# Autodesk Inventor assembly: Ensamble_Base_MX-28
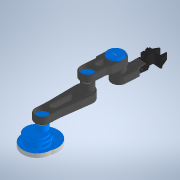
[picture p0: Inventor's stored thumbnail of the model, 180x180]
Saved by Autodesk Inventor 2021 (Build 250183000, 183)
## iProperties
Created: 2022-06-20
Part Number: Ensamble_Base_MX-28
Document SubType Name: Assembly
Designer: Alcatraz
Author: Alcatraz
## Documents named in this file (5)
- F:\Tesis\TESIS\Simulaciones\Movimiento en el plano\Base_MX-28\Ensamble_Base_MX-28.iam
- F:\Tesis\TESIS\Simulaciones\Base_MX28.ipt
- F:\Tesis\TESIS\Simulaciones\Eslabon_1.ipt
- F:\Tesis\TESIS\Simulaciones\Eslabon_2.ipt
- F:\Tesis\TESIS\Simulaciones\Eslabon_3.ipt
## Components (4 placed, 4 different names)
1. Base_MX28:1 — De rotación:1
2. Eslabon_1:1 — De rotación:1, De rotación:2
3. Eslabon_2:1 — De rotación:2, De rotación:3
4. Eslabon_3:1 — De rotación:3
## Relationships (3: RevoluteJoint 3)
- De rotación:1 [RevoluteJoint]: Base_MX28:1 ↔ Eslabon_1:1
- De rotación:2 [RevoluteJoint]: Eslabon_1:1 ↔ Eslabon_2:1
- De rotación:3 [RevoluteJoint]: Eslabon_2:1 ↔ Eslabon_3:1
